# Autodesk Inventor assembly: Assembly_base
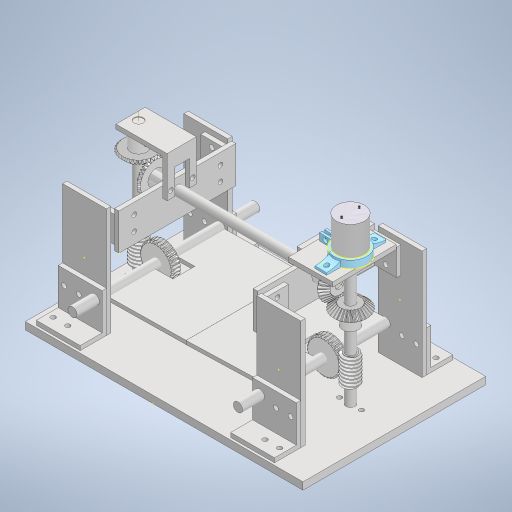
[picture p0: Inventor's stored thumbnail of the model, 512x512]
Saved by Autodesk Inventor 2023 (Build 270158000, 158)
## iProperties
Created: 2023-02-09
Part Number: Assembly_base
Document SubType Name: Assembly
Designer: deepa
Author: deepa
## Documents named in this file (19)
- C:\Users\deepa\OneDrive\Desktop\Courses\4thsem\ta220\Group 27 TA\Assembly_base.iam
- C:\Users\deepa\OneDrive\Desktop\Courses\4thsem\ta220\Group 27 TA\Base Plate.ipt
- C:\Users\deepa\OneDrive\Desktop\Courses\4thsem\ta220\Group 27 TA\Base_Connector1.ipt
- C:\Users\deepa\OneDrive\Desktop\Courses\4thsem\ta220\Group 27 TA\Base_Connector2.ipt
- C:\Users\deepa\OneDrive\Desktop\Courses\4thsem\ta220\Group 27 TA\Side_Plate1.ipt
- C:\Users\deepa\OneDrive\Desktop\Courses\4thsem\ta220\Group 27 TA\Side_plate2.ipt
- C:\Users\deepa\OneDrive\Desktop\Courses\4thsem\ta220\Group 27 TA\support plate 2.ipt
- C:\Users\deepa\OneDrive\Desktop\Courses\4thsem\ta220\Group 27 TA\Normal_Connector.ipt
- C:\Users\deepa\OneDrive\Desktop\Courses\4thsem\ta220\Group 27 TA\Assembly_base\Design Accelerator\Bevel Gears3.iam
- C:\Users\deepa\OneDrive\Desktop\Courses\4thsem\ta220\Group 27 TA\rod_250mm.ipt
- C:\Users\deepa\OneDrive\Desktop\Courses\4thsem\ta220\Group 27 TA\Assembly_base\Design Accelerator\Worm Gears7.iam
- C:\Users\deepa\OneDrive\Desktop\Courses\4thsem\ta220\Group 27 TA\sadak_.ipt
- C:\Users\deepa\OneDrive\Desktop\Courses\4thsem\ta220\Group 27 TA\motor.ipt
- C:\Users\deepa\OneDrive\Desktop\Courses\4thsem\ta220\Group 27 TA\motor_angle.ipt
- C:\Users\deepa\OneDrive\Desktop\Courses\4thsem\ta220\Group 27 TA\motor_base.ipt
- C:\Users\deepa\OneDrive\Desktop\Courses\4thsem\ta220\Group 27 TA\rod_130mm.ipt
- C:\Users\deepa\OneDrive\Desktop\Courses\4thsem\ta220\Group 27 TA\rod_195mm.ipt
- C:\Users\deepa\OneDrive\Desktop\Courses\4thsem\ta220\Group 27 TA\motor holder.ipt
- C:\Users\deepa\OneDrive\Desktop\Courses\4thsem\ta220\Group 27 TA\motor_angle - non motor.ipt
## Components (31 placed, 18 different names)
1. Base Plate:1 — Mate:1, Mate:2, Mate:3, Mate:4, Mate:5, Mate:6, Mate:7, Mate:8, Mate:9, Mate:10, Mate:11, Mate:12, Mate:13, Mate:14, Mate:15, Mate:16, Mate:21, Mate:106, Mate:112, Flush:8
2. Base_Connector1:1 — Mate:1, Mate:2, Mate:3, Mate:22, Mate:23
3. Base_Connector1:2 — Mate:4, Mate:5, Mate:6, Mate:26, Mate:32
4. Base_Connector2:1 — Mate:7, Mate:11, Mate:12, Mate:18, Mate:19, Mate:95
5. Base_Connector2:2 — Mate:8, Mate:9, Mate:10, Mate:24, Mate:25, Mate:92
6. Side_Plate1:1 — Mate:14, Mate:21, Mate:22, Mate:23, Mate:40, Flush:1, Mate:54, Mate:99
7. Side_plate2:1 — Mate:13, Mate:18, Mate:19, Flush:2, Mate:45, Mate:46, Mate:98
8. Side_Plate1:2 — Mate:15, Mate:24, Mate:25, Mate:39
9. Side_plate2:2 — Mate:16, Mate:26, Mate:32, Mate:57
10. support plate 2:1 — Mate:36, Mate:37, Mate:38, Mate:40, Flush:1, Mate:114, Mate:120, Mate:122
11. Normal_Connector:1 — Mate:36, Mate:38, Mate:39, Flush:5
12. Normal_Connector:2 — Mate:37, Mate:54, Flush:6
13. support plate 2:2 — Flush:2, Mate:46, Mate:58, Mate:100, Flush:7
14. Normal_Connector:3 — Mate:45, Flush:6
15. Normal_Connector:4 — Mate:57, Mate:58, Flush:5
16. Bevel Gears:4 [sub-assembly] — Mate:111, Mate:115
17. Bevel Gears:5 [sub-assembly] — Mate:109, Mate:113
18. rod_250mm:1 — Mate:95, Mate:96
19. rod_250mm:2 — Mate:92, Mate:97
20. Worm Gears:9 [sub-assembly]
21. Worm Gears:10 [sub-assembly] — Mate:107
22. sadak_:1 — Mate:96, Mate:98
23. sadak_:2 — Mate:97, Mate:99
24. motor:1 — Mate:104, Mate:105, Mate:118
25. motor_angle:1 — Mate:100, Mate:101, Mate:102, Flush:7
26. motor_base:1 — Mate:101, Mate:102, Mate:104, Mate:105, Mate:117
27. rod_130mm:1 — Mate:106, Mate:109, Flush:8, Mate:121
28. rod_195mm:1 — Mate:107, Mate:111, Mate:112, Mate:116, Mate:118
29. rod_250mm:3 — Mate:113, Mate:114, Mate:115
30. motor holder:1 — Mate:116, Mate:117
31. motor_angle - non motor:1 — Mate:120, Mate:121, Mate:122
## Relationships (68: Mate 62, Flush 6)
- Mate:1: Base Plate:1 ↔ Base_Connector1:1
- Mate:2: Base Plate:1 ↔ Base_Connector1:1
- Mate:3: Base Plate:1 ↔ Base_Connector1:1
- Mate:4: Base Plate:1 ↔ Base_Connector1:2
- Mate:5: Base Plate:1 ↔ Base_Connector1:2
- Mate:6: Base Plate:1 ↔ Base_Connector1:2
- Mate:7: Base Plate:1 ↔ Base_Connector2:1
- Mate:8: Base Plate:1 ↔ Base_Connector2:2
- Mate:9: Base Plate:1 ↔ Base_Connector2:2
- Mate:10: Base Plate:1 ↔ Base_Connector2:2
- Mate:11: Base Plate:1 ↔ Base_Connector2:1
- Mate:12: Base Plate:1 ↔ Base_Connector2:1
- Mate:13: Base Plate:1 ↔ Side_plate2:1
- Mate:14: Base Plate:1 ↔ Side_Plate1:1
- Mate:15: Base Plate:1 ↔ Side_Plate1:2
- Mate:16: Base Plate:1 ↔ Side_plate2:2
- Mate:18: Base_Connector2:1 ↔ Side_plate2:1
- Mate:19: Base_Connector2:1 ↔ Side_plate2:1
- Mate:21: Base Plate:1 ↔ Side_Plate1:1
- Mate:22: Base_Connector1:1 ↔ Side_Plate1:1
- Mate:23: Base_Connector1:1 ↔ Side_Plate1:1
- Mate:24: Base_Connector2:2 ↔ Side_Plate1:2
- Mate:25: Base_Connector2:2 ↔ Side_Plate1:2
- Mate:26: Base_Connector1:2 ↔ Side_plate2:2
- Mate:32: Base_Connector1:2 ↔ Side_plate2:2
- Mate:36: support plate 2:1 ↔ Normal_Connector:1
- Mate:37: support plate 2:1 ↔ Normal_Connector:2
- Mate:38: support plate 2:1 ↔ Normal_Connector:1
- Mate:39: Side_Plate1:2 ↔ Normal_Connector:1
- Mate:40 (5 mm): Side_Plate1:1 ↔ support plate 2:1
- Flush:1: Side_Plate1:1 ↔ support plate 2:1
- [Mate]: support plate 2:2 ↔ Normal_Connector:3
- [Mate]: support plate 2:2 ↔ Normal_Connector:3
- Flush:2: Side_plate2:1 ↔ support plate 2:2
- Mate:45: Side_plate2:1 ↔ Normal_Connector:3
- Mate:46 (5 mm): Side_plate2:1 ↔ support plate 2:2
- Mate:54: Side_Plate1:1 ↔ Normal_Connector:2
- Mate:57: Side_plate2:2 ↔ Normal_Connector:4
- Mate:58: support plate 2:2 ↔ Normal_Connector:4
- Flush:5: Normal_Connector:1 ↔ Normal_Connector:4
- Flush:6: Normal_Connector:2 ↔ Normal_Connector:3
- Mate:92: Base_Connector2:2 ↔ rod_250mm:2
- Mate:95: Base_Connector2:1 ↔ rod_250mm:1
- Mate:96: rod_250mm:1 ↔ sadak_:1
- Mate:97: rod_250mm:2 ↔ sadak_:2
- Mate:98: Side_plate2:1 ↔ sadak_:1
- Mate:99: Side_Plate1:1 ↔ sadak_:2
- Mate:100: support plate 2:2 ↔ motor_angle:1
- Mate:101: motor_angle:1 ↔ motor_base:1
- Mate:102: motor_angle:1 ↔ motor_base:1
- Mate:104: motor:1 ↔ motor_base:1
- Mate:105: motor:1 ↔ motor_base:1
- Mate:106: Base Plate:1 ↔ rod_130mm:1
- Mate:107: Worm Gears:10 ↔ rod_195mm:1
- Mate:109: Bevel Gears:5 ↔ rod_130mm:1
- Mate:111: Bevel Gears:4 ↔ rod_195mm:1
- Mate:112: Base Plate:1 ↔ rod_195mm:1
- Mate:113: Bevel Gears:5 ↔ rod_250mm:3
- Mate:114: support plate 2:1 ↔ rod_250mm:3
- Mate:115: Bevel Gears:4 ↔ rod_250mm:3
- Mate:116: rod_195mm:1 ↔ motor holder:1
- Mate:117: motor_base:1 ↔ motor holder:1
- Flush:7: support plate 2:2 ↔ motor_angle:1
- Mate:118: motor:1 ↔ rod_195mm:1
- Flush:8: Base Plate:1 ↔ rod_130mm:1
- Mate:120 (35 mm): support plate 2:1 ↔ motor_angle - non motor:1
- Mate:121: rod_130mm:1 ↔ motor_angle - non motor:1
- Mate:122: support plate 2:1 ↔ motor_angle - non motor:1
## Named parameters: d58_d50 = 0 mm, d60_d53 = 0 mm
